# Autodesk Inventor assembly: micromanipulator
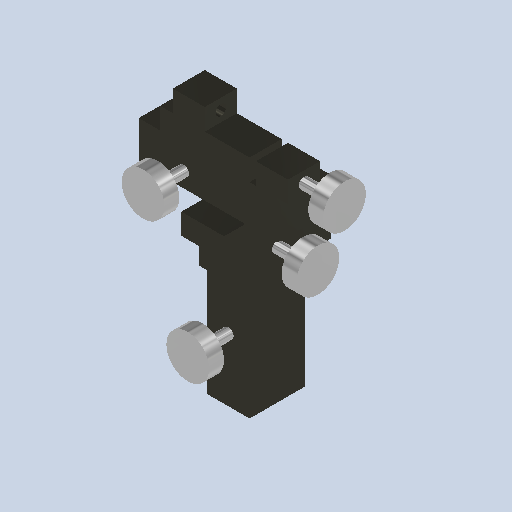
[picture p0: Inventor's stored thumbnail of the model, 512x512]
Saved by Autodesk Inventor 2024 (Build 280153000, 153)
## iProperties
Created: 2023-06-14
Part Number: micromanipulator
Document SubType Name: Assembly
Designer: dsdan
Author: dsdan
## Documents named in this file (3)
- E:\OneDrive - Imperial College London\DragonVision_DanielKo\Instrumentation\Ephys_rig_2021\micromanipulator.iam
- E:\OneDrive - Imperial College London\DragonVision_DanielKo\Instrumentation\Ephys_rig_2021\micromanipulator.ipt
- E:\OneDrive - Imperial College London\DragonVision_DanielKo\Instrumentation\Ephys_rig_2021\micromanipulator_knob.ipt
## Components (5 placed, 2 different names)
1. micromanipulator:1 — Mate:1, Mate:2, Mate:3, Mate:4, Mate:5, Mate:6, Mate:7, Mate:8
2. micromanipulator_knob:1 — Mate:1, Mate:2
3. micromanipulator_knob:2 — Mate:4, Mate:8
4. micromanipulator_knob:3 — Mate:3, Mate:6
5. micromanipulator_knob:4 — Mate:5, Mate:7
## Relationships (8: Mate 8)
- Mate:1: micromanipulator:1 ↔ micromanipulator_knob:1
- Mate:2: micromanipulator:1 ↔ micromanipulator_knob:1
- Mate:3: micromanipulator:1 ↔ micromanipulator_knob:3
- Mate:4: micromanipulator:1 ↔ micromanipulator_knob:2
- Mate:5: micromanipulator:1 ↔ micromanipulator_knob:4
- Mate:6: micromanipulator:1 ↔ micromanipulator_knob:3
- Mate:7: micromanipulator:1 ↔ micromanipulator_knob:4
- Mate:8: micromanipulator:1 ↔ micromanipulator_knob:2
